# Autodesk Inventor assembly: 2
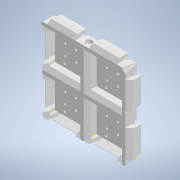
[picture p0: Inventor's stored thumbnail of the model, 180x180]
Saved by Autodesk Inventor 2021 (Build 250183000, 183)
## iProperties
Created: 2021-01-06
Part Number: 2
Document SubType Name: Assembly
Designer: Luke Kamols
Author: Luke Kamols
## Documents named in this file (6)
- C:\Users\Luke Kamols\Documents\GitHub\chess\Board\Pieces\2.iam
- C:\Users\Luke Kamols\Documents\GitHub\chess\Board\Components\base.iam
- C:\Users\Luke Kamols\Documents\GitHub\chess\Board\Components\inside-join-hole.iam
- C:\Users\Luke Kamols\Documents\GitHub\chess\Board\Components\inside-join-no-hole.iam
- C:\Users\Luke Kamols\Documents\GitHub\chess\Board\Components\outside-join-hole.iam
- C:\Users\Luke Kamols\Documents\GitHub\chess\Board\Components\outside-join-no-hole.iam
## Components (5 placed, 5 different names)
1. base:1 [sub-assembly] — Mate:1, Flush:1, Flush:2, Mate:2, Flush:3, Flush:4, Mate:3, Flush:5, Flush:6, Mate:4, Flush:7, Flush:8
2. inside-join-hole:1 [sub-assembly] — Mate:2, Flush:3, Flush:4
3. inside-join-no-hole:1 [sub-assembly] — Mate:3, Flush:5, Flush:6
4. outside-join-hole:1 [sub-assembly] — Mate:1, Flush:1, Flush:2
5. outside-join-no-hole:1 [sub-assembly] — Mate:4, Flush:7, Flush:8
## Relationships (12: Flush 8, Mate 4)
- Mate:1: base:1 ↔ outside-join-hole:1
- Flush:1: base:1 ↔ outside-join-hole:1
- Flush:2: base:1 ↔ outside-join-hole:1
- Mate:2: base:1 ↔ inside-join-hole:1
- Flush:3: base:1 ↔ inside-join-hole:1
- Flush:4: base:1 ↔ inside-join-hole:1
- Mate:3: base:1 ↔ inside-join-no-hole:1
- Flush:5: base:1 ↔ inside-join-no-hole:1
- Flush:6: base:1 ↔ inside-join-no-hole:1
- Mate:4: base:1 ↔ outside-join-no-hole:1
- Flush:7: base:1 ↔ outside-join-no-hole:1
- Flush:8: base:1 ↔ outside-join-no-hole:1
